# Autodesk Inventor assembly: chamber_assembly
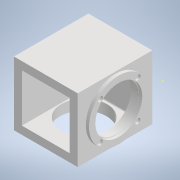
[picture p0: Inventor's stored thumbnail of the model, 180x180]
Saved by Autodesk Inventor 2021 (Build 250183000, 183)
## iProperties
Created: 2021-06-14
Part Number: chamber_assembly
Document SubType Name: Assembly
Designer: MicroscopyInnovation
Author: MicroscopyInnovation
## Documents named in this file (3)
- C:\Users\MicroscopyInnovation\Desktop\CAD\Microscopes\CTASLMv1\Workgroups\NotInProject\Components\Chamber\chamber_assembly.iam
- C:\Users\MicroscopyInnovation\Desktop\CAD\Microscopes\CTASLMv1\Workgroups\NotInProject\Components\Chamber\chamber.ipt
- C:\Users\MicroscopyInnovation\Desktop\CAD\Microscopes\CTASLMv1\Workgroups\NotInProject\Components\chamberPlateCircle.ipt
## Components (3 placed, 2 different names)
1. chamber:1 — Mate:1, Mate:2, Mate:3, Mate:4
2. chamberPlateCircle:1 — Mate:1, Mate:2
3. chamberPlateCircle:2 — Mate:3, Mate:4
## Relationships (4: Mate 4)
- Mate:1: chamber:1 ↔ chamberPlateCircle:1
- Mate:2: chamber:1 ↔ chamberPlateCircle:1
- Mate:3: chamber:1 ↔ chamberPlateCircle:2
- Mate:4: chamber:1 ↔ chamberPlateCircle:2
